# Autodesk Inventor assembly: RailAttachmentAssembly
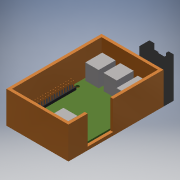
[picture p0: Inventor's stored thumbnail of the model, 180x180]
Saved by Autodesk Inventor 2018 (Build 220112000, 112)
## iProperties
Created: 2019-04-01
Part Number: RailAttachmentAssembly
Document SubType Name: Assembly
Designer: snipe
Author: snipe
## Documents named in this file (4)
- C:\Users\snipe\Documents\CPRE186-CAD\RailAttachmentAssembly.iam
- C:\Users\snipe\Documents\CPRE186-CAD\nerfRailMount.ipt
- C:\Users\snipe\Documents\CPRE186-CAD\Raspi3B+_Case.ipt
- C:\Users\snipe\Documents\CPRE186-CAD\Raspi3B+_Mockup.ipt
## Components (3 placed, 3 different names)
1. nerfRailMount:1 — Mate:1, Flush:1, Flush:2
2. Raspi3B+_Case:1 — Mate:1, Flush:1, Mate:2, Mate:3, Flush:2
3. Raspi3B+_Mockup:1 — Mate:2, Mate:3
## Relationships (5: Mate 3, Flush 2)
- Mate:1: nerfRailMount:1 ↔ Raspi3B+_Case:1
- Flush:1: nerfRailMount:1 ↔ Raspi3B+_Case:1
- Mate:2: Raspi3B+_Case:1 ↔ Raspi3B+_Mockup:1
- Mate:3: Raspi3B+_Case:1 ↔ Raspi3B+_Mockup:1
- Flush:2: nerfRailMount:1 ↔ Raspi3B+_Case:1
